# Autodesk Inventor assembly: 00_XY_stage-Chinese_60x60_R1
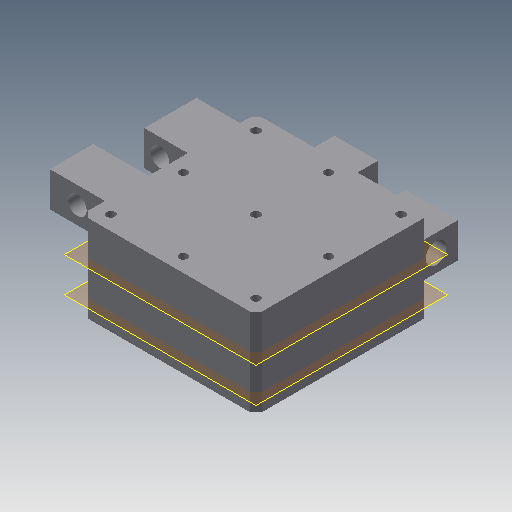
[picture p0: Inventor's stored thumbnail of the model, 512x512]
Saved by Autodesk Inventor 2019 (Build 230136000, 136)
## iProperties
Created: 2019-05-02
Part Number: 00_XY_stage-Chinese_60x60_R1
Document SubType Name: Assembly
Designer: diederichbenedict
Author: diederichbenedict
## Documents named in this file (4)
- C:\Users\diederichbenedict\Dropbox\Dokumente\Promotion\PROJECTS\STORMoChip\GITHUB\CAD\Nanoscopy-on-the-cheap\Workspace\00_XY_stage-Chinese_60x60_R1.iam
- C:\Users\diederichbenedict\Dropbox\Dokumente\Promotion\PROJECTS\STORMoChip\GITHUB\CAD\Nanoscopy-on-the-cheap\Workspace\00_XY_stage-Chinese_60x60-Top_R1.ipt
- C:\Users\diederichbenedict\Dropbox\Dokumente\Promotion\PROJECTS\STORMoChip\GITHUB\CAD\Nanoscopy-on-the-cheap\Workspace\00_XY_stage-Chinese_60x60-Middle_R1.ipt
- C:\Users\diederichbenedict\Dropbox\Dokumente\Promotion\PROJECTS\STORMoChip\GITHUB\CAD\Nanoscopy-on-the-cheap\Workspace\00_XY_stage-Chinese_60x60-Bottom_R1.ipt
## Components (3 placed, 3 different names)
1. 00_XY_stage-Chinese_60x60-Top_R1:1 — Flush:2, Flush:1
2. 00_XY_stage-Chinese_60x60-Middle_R1:1 — Flush:2, Flush:1, Flush:4, Flush:3
3. 00_XY_stage-Chinese_60x60-Bottom_R1:1 — Flush:4, Flush:3
## Relationships (4: Mate 4)
- Flush:2 [Mate]: 00_XY_stage-Chinese_60x60-Top_R1:1 ↔ 00_XY_stage-Chinese_60x60-Middle_R1:1
- Flush:1 [Mate]: 00_XY_stage-Chinese_60x60-Top_R1:1 ↔ 00_XY_stage-Chinese_60x60-Middle_R1:1
- Flush:4 [Mate]: 00_XY_stage-Chinese_60x60-Middle_R1:1 ↔ 00_XY_stage-Chinese_60x60-Bottom_R1:1
- Flush:3 [Mate]: 00_XY_stage-Chinese_60x60-Middle_R1:1 ↔ 00_XY_stage-Chinese_60x60-Bottom_R1:1
